# Autodesk Inventor assembly: Weight Applier for Modules v3
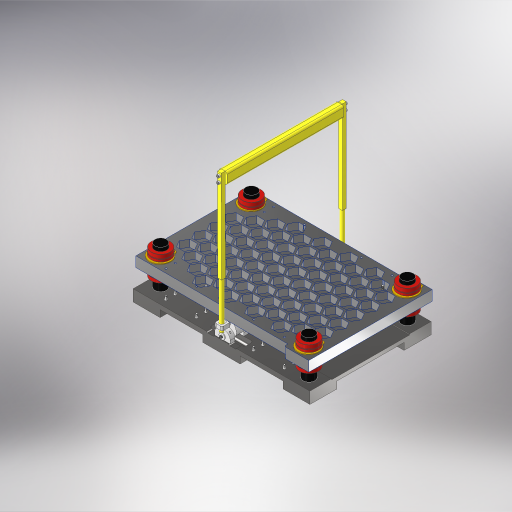
[picture p0: Inventor's stored thumbnail of the model, 512x512]
Saved by Autodesk Inventor 2024 (Build 280153000, 153)
## iProperties
Created: 2023-01-04
Part Number: Weight Applier for Modules v3
Document SubType Name: Assembly
Designer: Hayden Swanson
Author: Hayden Swanson
## Documents named in this file (12)
- C:\Users\cfang\Desktop\nebraska-silicon-lab\Hardware\ETL\Module Assembly\WAM_v4\Weight Applier for Modules v4.iam
- C:\Users\cfang\Desktop\nebraska-silicon-lab\Hardware\ETL\Module Assembly\WAM_v4\Rod.ipt
- C:\Users\cfang\Desktop\nebraska-silicon-lab\Hardware\ETL\Module Assembly\WAM_v4\Weight Frame Top.ipt
- C:\Users\cfang\Desktop\nebraska-silicon-lab\Hardware\ETL\Module Assembly\WAM_v4\Weight Frame.ipt
- C:\Users\cfang\Desktop\nebraska-silicon-lab\Hardware\ETL\Module Assembly\WAM_v4\90272A972_Zinc-Plated Steel Pan Head Phillips Screw.ipt
- C:\Users\cfang\Desktop\nebraska-silicon-lab\Hardware\ETL\Module Assembly\WAM_v4\90044A111_Black-Oxide Alloy Steel Socket Head Screw.ipt
- C:\Users\cfang\Desktop\nebraska-silicon-lab\Hardware\ETL\Module Assembly\WAM_v4\handle.ipt
- C:\Users\cfang\Desktop\nebraska-silicon-lab\Hardware\ETL\Module Assembly\WAM_v4\handle handle.ipt
- C:\Users\cfang\Desktop\nebraska-silicon-lab\Hardware\ETL\Module Assembly\WAM_v4\9533T5_Self-Aligning Linear Sleeve Bearing.ipt
- C:\Users\cfang\Desktop\nebraska-silicon-lab\Hardware\ETL\Module Assembly\WAM_v4\LockMechanism_v3.iam
- C:\Users\cfang\Desktop\nebraska-silicon-lab\Hardware\ETL\Module Assembly\WAM_v4\91590A137_External Retaining Ring.ipt
- C:\Users\cfang\Desktop\nebraska-silicon-lab\Hardware\ETL\Module Assembly\WAM_v4\9634K37_Extension Spring Stud Anchor.ipt
## Components (71 placed, 11 different names)
1. Weight Frame:1 — Mate:111, Mate:120, Mate:127, Mate:128, Mate:129, Mate:130, Mate:131, Mate:132, Mate:133, Mate:134, Mate:135, Mate:136, Mate:137, Mate:138, Mate:139, Mate:140, Mate:141, Mate:142, Mate:160, Mate:161, Mate:162, Mate:163, Mate:164, Mate:165, Mate:166, Mate:167, Mate:170, Mate:173, Mate:183, Mate:184, Mate:189, Mate:191, Insert:7, Insert:8, Insert:9, Insert:17, Insert:18, Insert:19, Insert:20, Insert:21, Insert:22, Insert:23, Insert:24, Insert:25, Insert:26, Insert:27, Insert:28
2. Weight Frame Top:2 — Mate:113, Mate:122, Mate:180, Mate:181, Mate:182, Mate:192, Flush:1, Mate:193, Flush:2, Flush:3, Insert:1, Insert:2, Insert:3, Insert:4, Insert:5, Insert:6, Insert:10, Insert:11, Insert:12, Insert:13, Insert:14, Insert:15, Insert:16, Insert:29, Insert:30, Insert:31, Insert:32, Insert:33, Insert:34, Insert:35, Insert:36
3. handle:1 — Mate:91, Mate:92, Mate:150, Mate:152, Mate:155, Mate:156, Mate:157, Mate:174
4. handle:2 — Mate:93, Mate:94, Mate:151, Mate:153, Mate:154, Mate:175
5. handle handle:1 — Mate:150, Mate:151, Mate:152, Mate:157
6. 90044A111_Black-Oxide Alloy Steel Socket Head Screw:13 — Mate:91, Mate:156
7. 90044A111_Black-Oxide Alloy Steel Socket Head Screw:14 — Mate:92, Mate:155
8. 90044A111_Black-Oxide Alloy Steel Socket Head Screw:15 — Mate:93, Mate:154
9. 90044A111_Black-Oxide Alloy Steel Socket Head Screw:16 — Mate:94, Mate:153
10. Rod:1 — Mate:111, Mate:113, Mate:124, Mate:186
11. Rod:4 — Mate:120, Mate:122, Mate:123, Mate:185
12. 9533T5_Self-Aligning Linear Sleeve Bearing:1 — Mate:123, Flush:2
13. 9533T5_Self-Aligning Linear Sleeve Bearing:2 — Mate:124, Mate:176, Mate:177, Mate:178, Mate:179
14. 9533T5_Self-Aligning Linear Sleeve Bearing:3 — Mate:187, Flush:1
15. 90272A972_Zinc-Plated Steel Pan Head Phillips Screw:1 — Mate:166, Mate:167, Mate:187, Mate:188
16. 90272A972_Zinc-Plated Steel Pan Head Phillips Screw:2 — Mate:160, Mate:161, Mate:190
17. 90272A972_Zinc-Plated Steel Pan Head Phillips Screw:3 — Mate:162, Mate:163, Mate:185
18. 90044A111_Black-Oxide Alloy Steel Socket Head Screw:17 — Mate:127, Mate:132
19. 90044A111_Black-Oxide Alloy Steel Socket Head Screw:18 — Mate:129, Mate:131, Mate:169
20. 90044A111_Black-Oxide Alloy Steel Socket Head Screw:19 — Mate:130, Mate:133
21. 90044A111_Black-Oxide Alloy Steel Socket Head Screw:20 — Mate:128, Mate:134, Mate:168
22. 90044A111_Black-Oxide Alloy Steel Socket Head Screw:21 — Mate:135, Mate:141
23. 90044A111_Black-Oxide Alloy Steel Socket Head Screw:22 — Mate:136, Mate:142, Mate:171
24. 90044A111_Black-Oxide Alloy Steel Socket Head Screw:23 — Mate:137, Mate:140, Mate:172
25. 90044A111_Black-Oxide Alloy Steel Socket Head Screw:24 — Mate:138, Mate:139
26. 90272A972_Zinc-Plated Steel Pan Head Phillips Screw:4 — Mate:164, Mate:165, Mate:186
27. LockMechanism_v3:1 [sub-assembly] — Mate:168, Mate:169, Mate:170, Mate:175
28. LockMechanism_v3:2 [sub-assembly] — Mate:171, Mate:172, Mate:173, Mate:174, Mate:193
29. 91590A137_External Retaining Ring:1 — Mate:176, Mate:177
30. 91590A137_External Retaining Ring:2 — Mate:178, Mate:179, Mate:180
31. 9634K37_Extension Spring Stud Anchor:1 — Mate:181, Mate:182
32. 9634K37_Extension Spring Stud Anchor:2 — Mate:183, Mate:184
33. Rod:5 — Mate:188, Mate:189
34. Rod:6 — Mate:190, Mate:191
35. 9533T5_Self-Aligning Linear Sleeve Bearing:4 — Mate:192, Flush:3
36. 91590A137_External Retaining Ring:3 — Insert:1
37. 91590A137_External Retaining Ring:4 — Insert:2
38. 91590A137_External Retaining Ring:5 — Insert:3
39. 91590A137_External Retaining Ring:6 — Insert:4
40. 91590A137_External Retaining Ring:7 — Insert:5
41. 91590A137_External Retaining Ring:8 — Insert:6
42. 9634K37_Extension Spring Stud Anchor:3 — Insert:7
43. 9634K37_Extension Spring Stud Anchor:4 — Insert:8
44. 9634K37_Extension Spring Stud Anchor:5 — Insert:9
45. 9634K37_Extension Spring Stud Anchor:6 — Insert:10
46. 9634K37_Extension Spring Stud Anchor:7 — Insert:11
47. 9634K37_Extension Spring Stud Anchor:8 — Insert:12
48. 9634K37_Extension Spring Stud Anchor:9 — Insert:13
49. 9634K37_Extension Spring Stud Anchor:10 — Insert:14
50. 9634K37_Extension Spring Stud Anchor:11 — Insert:15
51. 9634K37_Extension Spring Stud Anchor:12 — Insert:16
52. 9634K37_Extension Spring Stud Anchor:13 — Insert:17
53. 9634K37_Extension Spring Stud Anchor:14 — Insert:18
54. 9634K37_Extension Spring Stud Anchor:15 — Insert:19
55. 9634K37_Extension Spring Stud Anchor:16 — Insert:20
56. 9634K37_Extension Spring Stud Anchor:17 — Insert:21
57. 9634K37_Extension Spring Stud Anchor:18 — Insert:22
58. 9634K37_Extension Spring Stud Anchor:19 — Insert:23
59. 9634K37_Extension Spring Stud Anchor:20 — Insert:24
60. 9634K37_Extension Spring Stud Anchor:21 — Insert:25
61. 9634K37_Extension Spring Stud Anchor:22 — Insert:26
62. 9634K37_Extension Spring Stud Anchor:23 — Insert:27
63. 9634K37_Extension Spring Stud Anchor:24 — Insert:28
64. 9634K37_Extension Spring Stud Anchor:25 — Insert:29
65. 9634K37_Extension Spring Stud Anchor:26 — Insert:30
66. 9634K37_Extension Spring Stud Anchor:27 — Insert:31
67. 9634K37_Extension Spring Stud Anchor:28 — Insert:32
68. 9634K37_Extension Spring Stud Anchor:29 — Insert:33
69. 9634K37_Extension Spring Stud Anchor:30 — Insert:34
70. 9634K37_Extension Spring Stud Anchor:31 — Insert:35
71. 9634K37_Extension Spring Stud Anchor:32 — Insert:36
## Relationships (107: Mate 68, Insert 36, Flush 3)
- Mate:91: handle:1 ↔ 90044A111_Black-Oxide Alloy Steel Socket Head Screw:13
- Mate:92: handle:1 ↔ 90044A111_Black-Oxide Alloy Steel Socket Head Screw:14
- Mate:93: handle:2 ↔ 90044A111_Black-Oxide Alloy Steel Socket Head Screw:15
- Mate:94: handle:2 ↔ 90044A111_Black-Oxide Alloy Steel Socket Head Screw:16
- Mate:111: Weight Frame:1 ↔ Rod:1
- Mate:113: Weight Frame Top:2 ↔ Rod:1
- Mate:120: Weight Frame:1 ↔ Rod:4
- Mate:122: Weight Frame Top:2 ↔ Rod:4
- Mate:123: Rod:4 ↔ 9533T5_Self-Aligning Linear Sleeve Bearing:1
- Mate:124: Rod:1 ↔ 9533T5_Self-Aligning Linear Sleeve Bearing:2
- Mate:127: Weight Frame:1 ↔ 90044A111_Black-Oxide Alloy Steel Socket Head Screw:17
- Mate:128: Weight Frame:1 ↔ 90044A111_Black-Oxide Alloy Steel Socket Head Screw:20
- Mate:129: Weight Frame:1 ↔ 90044A111_Black-Oxide Alloy Steel Socket Head Screw:18
- Mate:130: Weight Frame:1 ↔ 90044A111_Black-Oxide Alloy Steel Socket Head Screw:19
- Mate:131: Weight Frame:1 ↔ 90044A111_Black-Oxide Alloy Steel Socket Head Screw:18
- Mate:132: Weight Frame:1 ↔ 90044A111_Black-Oxide Alloy Steel Socket Head Screw:17
- Mate:133: Weight Frame:1 ↔ 90044A111_Black-Oxide Alloy Steel Socket Head Screw:19
- Mate:134: Weight Frame:1 ↔ 90044A111_Black-Oxide Alloy Steel Socket Head Screw:20
- Mate:135: Weight Frame:1 ↔ 90044A111_Black-Oxide Alloy Steel Socket Head Screw:21
- Mate:136: Weight Frame:1 ↔ 90044A111_Black-Oxide Alloy Steel Socket Head Screw:22
- Mate:137: Weight Frame:1 ↔ 90044A111_Black-Oxide Alloy Steel Socket Head Screw:23
- Mate:138: Weight Frame:1 ↔ 90044A111_Black-Oxide Alloy Steel Socket Head Screw:24
- Mate:139: Weight Frame:1 ↔ 90044A111_Black-Oxide Alloy Steel Socket Head Screw:24
- Mate:140: Weight Frame:1 ↔ 90044A111_Black-Oxide Alloy Steel Socket Head Screw:23
- Mate:141: Weight Frame:1 ↔ 90044A111_Black-Oxide Alloy Steel Socket Head Screw:21
- Mate:142: Weight Frame:1 ↔ 90044A111_Black-Oxide Alloy Steel Socket Head Screw:22
- Mate:150: handle:1 ↔ handle handle:1
- Mate:151: handle:2 ↔ handle handle:1
- Mate:152: handle:1 ↔ handle handle:1
- Mate:153: handle:2 ↔ 90044A111_Black-Oxide Alloy Steel Socket Head Screw:16
- Mate:154: handle:2 ↔ 90044A111_Black-Oxide Alloy Steel Socket Head Screw:15
- Mate:155: handle:1 ↔ 90044A111_Black-Oxide Alloy Steel Socket Head Screw:14
- Mate:156: handle:1 ↔ 90044A111_Black-Oxide Alloy Steel Socket Head Screw:13
- Mate:157: handle:1 ↔ handle handle:1
- Mate:160: Weight Frame:1 ↔ 90272A972_Zinc-Plated Steel Pan Head Phillips Screw:2
- Mate:161: Weight Frame:1 ↔ 90272A972_Zinc-Plated Steel Pan Head Phillips Screw:2
- Mate:162: Weight Frame:1 ↔ 90272A972_Zinc-Plated Steel Pan Head Phillips Screw:3
- Mate:163: Weight Frame:1 ↔ 90272A972_Zinc-Plated Steel Pan Head Phillips Screw:3
- Mate:164: Weight Frame:1 ↔ 90272A972_Zinc-Plated Steel Pan Head Phillips Screw:4
- Mate:165: Weight Frame:1 ↔ 90272A972_Zinc-Plated Steel Pan Head Phillips Screw:4
- Mate:166: Weight Frame:1 ↔ 90272A972_Zinc-Plated Steel Pan Head Phillips Screw:1
- Mate:167: Weight Frame:1 ↔ 90272A972_Zinc-Plated Steel Pan Head Phillips Screw:1
- Mate:168: 90044A111_Black-Oxide Alloy Steel Socket Head Screw:20 ↔ LockMechanism_v3:1
- Mate:169: 90044A111_Black-Oxide Alloy Steel Socket Head Screw:18 ↔ LockMechanism_v3:1
- Mate:170: Weight Frame:1 ↔ LockMechanism_v3:1
- Mate:171: 90044A111_Black-Oxide Alloy Steel Socket Head Screw:22 ↔ LockMechanism_v3:2
- Mate:172: 90044A111_Black-Oxide Alloy Steel Socket Head Screw:23 ↔ LockMechanism_v3:2
- Mate:173: Weight Frame:1 ↔ LockMechanism_v3:2
- Mate:174: handle:1 ↔ LockMechanism_v3:2
- Mate:175: handle:2 ↔ LockMechanism_v3:1
- Mate:176: 9533T5_Self-Aligning Linear Sleeve Bearing:2 ↔ 91590A137_External Retaining Ring:1
- Mate:177: 9533T5_Self-Aligning Linear Sleeve Bearing:2 ↔ 91590A137_External Retaining Ring:1
- Mate:178: 9533T5_Self-Aligning Linear Sleeve Bearing:2 ↔ 91590A137_External Retaining Ring:2
- Mate:179: 9533T5_Self-Aligning Linear Sleeve Bearing:2 ↔ 91590A137_External Retaining Ring:2
- Mate:180: Weight Frame Top:2 ↔ 91590A137_External Retaining Ring:2
- Mate:181: Weight Frame Top:2 ↔ 9634K37_Extension Spring Stud Anchor:1
- Mate:182: Weight Frame Top:2 ↔ 9634K37_Extension Spring Stud Anchor:1
- Mate:183: Weight Frame:1 ↔ 9634K37_Extension Spring Stud Anchor:2
- Mate:184: Weight Frame:1 ↔ 9634K37_Extension Spring Stud Anchor:2
- Mate:185: Rod:4 ↔ 90272A972_Zinc-Plated Steel Pan Head Phillips Screw:3
- Mate:186: Rod:1 ↔ 90272A972_Zinc-Plated Steel Pan Head Phillips Screw:4
- Mate:187: 9533T5_Self-Aligning Linear Sleeve Bearing:3 ↔ 90272A972_Zinc-Plated Steel Pan Head Phillips Screw:1
- Mate:188: 90272A972_Zinc-Plated Steel Pan Head Phillips Screw:1 ↔ Rod:5
- Mate:189: Weight Frame:1 ↔ Rod:5
- Mate:190: 90272A972_Zinc-Plated Steel Pan Head Phillips Screw:2 ↔ Rod:6
- Mate:191: Weight Frame:1 ↔ Rod:6
- Mate:192: Weight Frame Top:2 ↔ 9533T5_Self-Aligning Linear Sleeve Bearing:4
- Flush:1: Weight Frame Top:2 ↔ 9533T5_Self-Aligning Linear Sleeve Bearing:3
- Mate:193: Weight Frame Top:2 ↔ LockMechanism_v3:2
- Flush:2: Weight Frame Top:2 ↔ 9533T5_Self-Aligning Linear Sleeve Bearing:1
- Flush:3: Weight Frame Top:2 ↔ 9533T5_Self-Aligning Linear Sleeve Bearing:4
- Insert:1: Weight Frame Top:2 ↔ 91590A137_External Retaining Ring:3
- Insert:2: Weight Frame Top:2 ↔ 91590A137_External Retaining Ring:4
- Insert:3: Weight Frame Top:2 ↔ 91590A137_External Retaining Ring:5
- Insert:4: Weight Frame Top:2 ↔ 91590A137_External Retaining Ring:6
- Insert:5: Weight Frame Top:2 ↔ 91590A137_External Retaining Ring:7
- Insert:6: Weight Frame Top:2 ↔ 91590A137_External Retaining Ring:8
- Insert:7: Weight Frame:1 ↔ 9634K37_Extension Spring Stud Anchor:3
- Insert:8: Weight Frame:1 ↔ 9634K37_Extension Spring Stud Anchor:4
- Insert:9: Weight Frame:1 ↔ 9634K37_Extension Spring Stud Anchor:5
- Insert:10: Weight Frame Top:2 ↔ 9634K37_Extension Spring Stud Anchor:6
- Insert:11: Weight Frame Top:2 ↔ 9634K37_Extension Spring Stud Anchor:7
- Insert:12: Weight Frame Top:2 ↔ 9634K37_Extension Spring Stud Anchor:8
- Insert:13: Weight Frame Top:2 ↔ 9634K37_Extension Spring Stud Anchor:9
- Insert:14: Weight Frame Top:2 ↔ 9634K37_Extension Spring Stud Anchor:10
- Insert:15: Weight Frame Top:2 ↔ 9634K37_Extension Spring Stud Anchor:11
- Insert:16: Weight Frame Top:2 ↔ 9634K37_Extension Spring Stud Anchor:12
- Insert:17: Weight Frame:1 ↔ 9634K37_Extension Spring Stud Anchor:13
- Insert:18: Weight Frame:1 ↔ 9634K37_Extension Spring Stud Anchor:14
- Insert:19: Weight Frame:1 ↔ 9634K37_Extension Spring Stud Anchor:15
- Insert:20: Weight Frame:1 ↔ 9634K37_Extension Spring Stud Anchor:16
- Insert:21: Weight Frame:1 ↔ 9634K37_Extension Spring Stud Anchor:17
- Insert:22: Weight Frame:1 ↔ 9634K37_Extension Spring Stud Anchor:18
- Insert:23: Weight Frame:1 ↔ 9634K37_Extension Spring Stud Anchor:19
- Insert:24: Weight Frame:1 ↔ 9634K37_Extension Spring Stud Anchor:20
- Insert:25: Weight Frame:1 ↔ 9634K37_Extension Spring Stud Anchor:21
- Insert:26: Weight Frame:1 ↔ 9634K37_Extension Spring Stud Anchor:22
- Insert:27: Weight Frame:1 ↔ 9634K37_Extension Spring Stud Anchor:23
- Insert:28: Weight Frame:1 ↔ 9634K37_Extension Spring Stud Anchor:24
- Insert:29: Weight Frame Top:2 ↔ 9634K37_Extension Spring Stud Anchor:25
- Insert:30: Weight Frame Top:2 ↔ 9634K37_Extension Spring Stud Anchor:26
- Insert:31: Weight Frame Top:2 ↔ 9634K37_Extension Spring Stud Anchor:27
- Insert:32: Weight Frame Top:2 ↔ 9634K37_Extension Spring Stud Anchor:28
- Insert:33: Weight Frame Top:2 ↔ 9634K37_Extension Spring Stud Anchor:29
- Insert:34: Weight Frame Top:2 ↔ 9634K37_Extension Spring Stud Anchor:30
- Insert:35: Weight Frame Top:2 ↔ 9634K37_Extension Spring Stud Anchor:31
- Insert:36: Weight Frame Top:2 ↔ 9634K37_Extension Spring Stud Anchor:32
